# Autodesk Inventor assembly: SP16-2P female waterproof connector
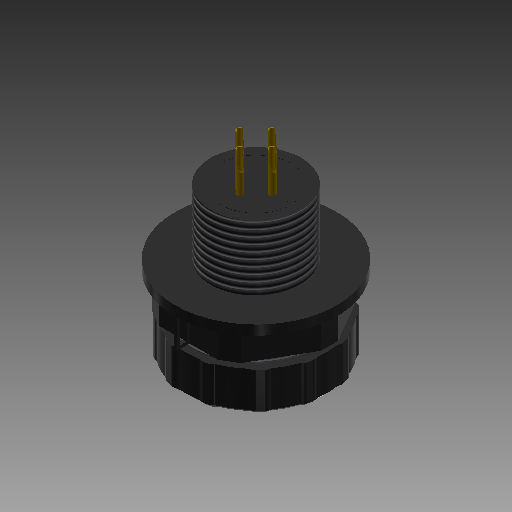
[picture p0: Inventor's stored thumbnail of the model, 512x512]
Saved by Autodesk Inventor 2018 (Build 220112000, 112)
## iProperties
Created: 2019-04-16
Part Number: SP16-2P female waterproof connector
Document SubType Name: Assembly
Designer: ZEUSLAP
Author: ZEUSLAP
## Documents named in this file (4)
- C:\Users\ZEUSLAP\YandexDisk\Inventor\SP16 waterproof connector\SP16-4P, female, back nut type.iam
- C:\Users\ZEUSLAP\YandexDisk\Inventor\SP16 waterproof connector\parts\cap.ipt
- C:\Users\ZEUSLAP\YandexDisk\Inventor\SP16 waterproof connector\parts\body.ipt
- C:\Users\ZEUSLAP\YandexDisk\Inventor\SP16 waterproof connector\parts\center_4p_female.iam
## Components (3 placed, 3 different names)
1. cap:1 — Mate:1, Mate:2, Mate:7
2. body:1 — Mate:1, Mate:2, Angle:1, Mate:8, Mate:9, Flush:1
3. center_4p_female:1 [sub-assembly] — Mate:8, Mate:9, Flush:1
## Relationships (7: Mate 5, Angle 1, Flush 1)
- Mate:1: cap:1 ↔ body:1
- Mate:2: cap:1 ↔ body:1
- Mate:7: cap:1
- Angle:1 (180 deg): body:1
- Mate:8: body:1 ↔ center_4p_female:1
- Mate:9: body:1 ↔ center_4p_female:1
- Flush:1: body:1 ↔ center_4p_female:1
